# Autodesk Inventor assembly: Drive Axle
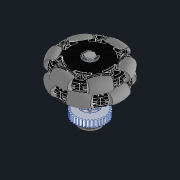
[picture p0: Inventor's stored thumbnail of the model, 180x180]
Saved by Autodesk Inventor 2022 (Build 260153000, 153)
## iProperties
Created: 2022-09-06
Part Number: Drive Axle
Document SubType Name: Assembly
Designer: robpl
Author: robpl
## Documents named in this file (11)
- C:\Users\robpl\OneDrive\Documents\Inventor\2022 FRC Season\Best Coast Drive\Drive Shaft.iam
- C:\Users\robpl\OneDrive\Documents\Inventor\2022 FRC Season\CAD Library\0.5 Flanged Hex Bearing (1.125 OD) (217-3875).ipt
- C:\Users\robpl\OneDrive\Documents\Inventor\2022 FRC Season\Best Coast Drive\36T Aluminum Spur Gear (20 DP, 1_2_ Hex Bore) (217-3214).ipt
- C:\Users\robpl\OneDrive\Documents\Inventor\2022 FRC Season\Best Coast Drive\0.5 Flanged Hex Bearing (1.125 OD) (217-3875).ipt
- C:\Users\robpl\OneDrive\Documents\Inventor\2022 FRC Season\WCD PnG 16012022-20220119T154132Z-001\WCD PnG 16012022\Workspaces\Workspace\12T Aluminum Hub Sprocket (#35 Chain, 1_2_ Hex Bore) (217-2662).ipt
- C:\Users\robpl\OneDrive\Documents\Inventor\2022 FRC Season\Best Coast Drive\Omni Wheel Axle.ipt
- C:\Users\robpl\OneDrive\Documents\Inventor\2022 FRC Season\Best Coast Drive\Omni Wheel\4_ Omni-Directional Wheel v2 (276-6194).iam
- C:\Users\robpl\OneDrive\Documents\Inventor\2022 FRC Season\Best Coast Drive\3mm 0.5in Hex Spacer.ipt
- C:\Users\robpl\OneDrive\Documents\Inventor\2022 FRC Season\Best Coast Drive\4.5mm 0.5in Hex Spacer.ipt
- C:\Users\robpl\OneDrive\Documents\Inventor\2022 FRC Season\Best Coast Drive\10mm E-Clip.ipt
- C:\Users\robpl\OneDrive\Documents\Inventor\2022 FRC Season\1mm 0.5in Hex Spacer.ipt
## Components (12 placed, 9 different names)
1. Omni Wheel Axle:1 — Mate:12, Mate:13, Mate:14, Mate:15, Mate:16, Mate:17, Mate:18, Mate:19, Flush:1, Mate:20, Mate:21, Flush:2, Flush:3, Mate:28, Mate:29, Mate:30, Mate:31, Mate:32, Mate:33
2. 0.5 Flanged Hex Bearing (1.125 OD) (217-3875):1 — Mate:12, Mate:13, Flush:1, Mate:23
3. 36T Aluminum Spur Gear (20 DP, 1_2_ Hex Bore) (217-3214):1 — Mate:18, Mate:19, Mate:23
4. 0.5 Flanged Hex Bearing (1.125 OD) (217-3875):2 — Mate:14, Mate:15, Mate:22, Flush:3, Mate:27
5. 12T Aluminum Hub Sprocket (#35 Chain, 1_2_ Hex Bore) (217-2662):1 — Mate:16, Mate:17, Mate:22, Mate:24, Mate:25, Mate:34, Mate:35
6. 4_ Omni-Directional Wheel v2 (276-6194):1 [sub-assembly] — Mate:20, Mate:21, Flush:2, Mate:26
7. 3mm 0.5in Hex Spacer:1 — Mate:24, Mate:25
8. 4.5mm 0.5in Hex Spacer:1 — Mate:26, Mate:27
9. 10mm E-Clip:1 — Mate:28, Mate:29
10. 10mm E-Clip:2 — Mate:32, Mate:33
11. 10mm E-Clip:3 — Mate:30, Mate:31
12. 1mm 0.5in Hex Spacer:1 — Mate:34, Mate:35
## Relationships (27: Mate 24, Flush 3)
- Mate:12: Omni Wheel Axle:1 ↔ 0.5 Flanged Hex Bearing (1.125 OD) (217-3875):1
- Mate:13: Omni Wheel Axle:1 ↔ 0.5 Flanged Hex Bearing (1.125 OD) (217-3875):1
- Mate:14: Omni Wheel Axle:1 ↔ 0.5 Flanged Hex Bearing (1.125 OD) (217-3875):2
- Mate:15: Omni Wheel Axle:1 ↔ 0.5 Flanged Hex Bearing (1.125 OD) (217-3875):2
- Mate:16: Omni Wheel Axle:1 ↔ 12T Aluminum Hub Sprocket (#35 Chain, 1_2_ Hex Bore) (217-2662):1
- Mate:17: Omni Wheel Axle:1 ↔ 12T Aluminum Hub Sprocket (#35 Chain, 1_2_ Hex Bore) (217-2662):1
- Mate:18: Omni Wheel Axle:1 ↔ 36T Aluminum Spur Gear (20 DP, 1_2_ Hex Bore) (217-3214):1
- Mate:19: Omni Wheel Axle:1 ↔ 36T Aluminum Spur Gear (20 DP, 1_2_ Hex Bore) (217-3214):1
- Flush:1: Omni Wheel Axle:1 ↔ 0.5 Flanged Hex Bearing (1.125 OD) (217-3875):1
- Mate:20: Omni Wheel Axle:1 ↔ 4_ Omni-Directional Wheel v2 (276-6194):1
- Mate:21: Omni Wheel Axle:1 ↔ 4_ Omni-Directional Wheel v2 (276-6194):1
- Flush:2: Omni Wheel Axle:1 ↔ 4_ Omni-Directional Wheel v2 (276-6194):1
- Mate:22 (3 mm): 0.5 Flanged Hex Bearing (1.125 OD) (217-3875):2 ↔ 12T Aluminum Hub Sprocket (#35 Chain, 1_2_ Hex Bore) (217-2662):1
- Mate:23: 0.5 Flanged Hex Bearing (1.125 OD) (217-3875):1 ↔ 36T Aluminum Spur Gear (20 DP, 1_2_ Hex Bore) (217-3214):1
- Flush:3: Omni Wheel Axle:1 ↔ 0.5 Flanged Hex Bearing (1.125 OD) (217-3875):2
- Mate:24: 12T Aluminum Hub Sprocket (#35 Chain, 1_2_ Hex Bore) (217-2662):1 ↔ 3mm 0.5in Hex Spacer:1
- Mate:25: 12T Aluminum Hub Sprocket (#35 Chain, 1_2_ Hex Bore) (217-2662):1 ↔ 3mm 0.5in Hex Spacer:1
- Mate:26: 4_ Omni-Directional Wheel v2 (276-6194):1 ↔ 4.5mm 0.5in Hex Spacer:1
- Mate:27: 0.5 Flanged Hex Bearing (1.125 OD) (217-3875):2 ↔ 4.5mm 0.5in Hex Spacer:1
- Mate:28: Omni Wheel Axle:1 ↔ 10mm E-Clip:1
- Mate:29: Omni Wheel Axle:1 ↔ 10mm E-Clip:1
- Mate:30: Omni Wheel Axle:1 ↔ 10mm E-Clip:3
- Mate:31: Omni Wheel Axle:1 ↔ 10mm E-Clip:3
- Mate:32: Omni Wheel Axle:1 ↔ 10mm E-Clip:2
- Mate:33: Omni Wheel Axle:1 ↔ 10mm E-Clip:2
- Mate:34: 12T Aluminum Hub Sprocket (#35 Chain, 1_2_ Hex Bore) (217-2662):1 ↔ 1mm 0.5in Hex Spacer:1
- Mate:35: 12T Aluminum Hub Sprocket (#35 Chain, 1_2_ Hex Bore) (217-2662):1 ↔ 1mm 0.5in Hex Spacer:1
